# Autodesk Inventor assembly: MG_996R
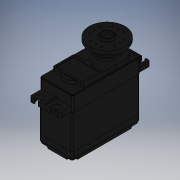
[picture p0: Inventor's stored thumbnail of the model, 180x180]
Saved by Autodesk Inventor 2016 (Build 200138000, 138)
## iProperties
Created: 2016-09-26
Part Number: MG_996R
Document SubType Name: Assembly
Designer: Julian
Author: Julian
## Documents named in this file (6)
- D:\Universidad\6 Semestre\Principios de Robotica\Proyeto de Semestre\MG996R\MG_996R.iam
- D:\Universidad\6 Semestre\Principios de Robotica\Proyeto de Semestre\MG996R\Base.ipt
- D:\Universidad\6 Semestre\Principios de Robotica\Proyeto de Semestre\MG996R\Medio.ipt
- D:\Universidad\6 Semestre\Principios de Robotica\Proyeto de Semestre\MG996R\Top.ipt
- D:\Universidad\6 Semestre\Principios de Robotica\Proyeto de Semestre\MG996R\Eje.ipt
- D:\Universidad\6 Semestre\Principios de Robotica\Proyeto de Semestre\MG996R\Acople circular.ipt
## Components (5 placed, 5 different names)
1. Top:1 — Rígido:2, De rotación:1
2. Medio:1 — Rígido:1, Rígido:2
3. Base:1 — Rígido:1
4. Eje:1 — De rotación:1, De rotación:2
5. Acople circular:1 — De rotación:2
## Relationships (4: WeldJoint 2, RevoluteJoint 2)
- Rígido:1 [WeldJoint]: Medio:1 ↔ Base:1
- Rígido:2 [WeldJoint]: Top:1 ↔ Medio:1
- De rotación:1 [RevoluteJoint]: Top:1 ↔ Eje:1
- De rotación:2 [RevoluteJoint]: Eje:1 ↔ Acople circular:1
